# Autodesk Inventor assembly: assembled-feed
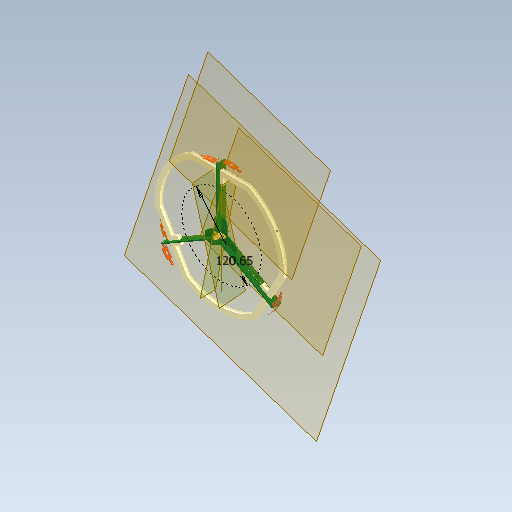
[picture p0: Inventor's stored thumbnail of the model, 512x512]
Saved by Autodesk Inventor 2021 (Build 250183000, 183)
## iProperties
Created: 2020-09-03
Part Number: assembled-feed
Document SubType Name: Assembly
Designer: dsouthall
Author: dsouthall
## Documents named in this file (4)
- C:\Users\dsouthall\OneDrive - The University of Chicago\Hpol\hpol-prototype\design\Model 8 in\assembled-feed.iam
- C:\Users\dsouthall\OneDrive - The University of Chicago\Hpol\hpol-prototype\design\Model 8 in\source\hub\tri-slot-hub.iam
- C:\Users\dsouthall\OneDrive - The University of Chicago\Hpol\hpol-prototype\design\Model 8 in\assembled-feed_feedline_8in.iam
- C:\Users\dsouthall\OneDrive - The University of Chicago\Hpol\hpol-prototype\design\Model 8 in\source\insert_8in.ipt
## Components (7 placed, 3 different names)
1. tri-slot-hub:1 [sub-assembly] — Mate:10, Angle:1, Mate:17, Mate:20, Mate:21, Mate:22, Mate:23, Mate:24, Mate:25, Mate:26, Mate:27, Mate:28, Mate:29, Mate:30
2. assembled-feed_feedline_8in:1 [sub-assembly] — Mate:21, Mate:22, Mate:23, Insert:4, Insert:6
3. assembled-feed_feedline_8in:2 [sub-assembly] — Mate:24, Mate:25, Mate:26, Insert:1, Insert:5
4. assembled-feed_feedline_8in:3 [sub-assembly] — Mate:27, Mate:28, Mate:29, Insert:2, Insert:3
5. insert_8in:1 — Insert:5, Insert:6
6. insert_8in:2 — Insert:1, Insert:2
7. insert_8in:3 — Insert:3, Insert:4
## Relationships (21: Mate 13, Insert 6, Angle 1, Flush 1)
- Mate:10: tri-slot-hub:1
- Angle:1 (0 deg): tri-slot-hub:1
- Mate:17: tri-slot-hub:1
- Mate:20: tri-slot-hub:1
- Flush:1 (-3.9973 mm)
- Mate:21: tri-slot-hub:1 ↔ assembled-feed_feedline_8in:1
- Mate:22: tri-slot-hub:1 ↔ assembled-feed_feedline_8in:1
- Mate:23: tri-slot-hub:1 ↔ assembled-feed_feedline_8in:1
- Mate:24: tri-slot-hub:1 ↔ assembled-feed_feedline_8in:2
- Mate:25: tri-slot-hub:1 ↔ assembled-feed_feedline_8in:2
- Mate:26: tri-slot-hub:1 ↔ assembled-feed_feedline_8in:2
- Mate:27: tri-slot-hub:1 ↔ assembled-feed_feedline_8in:3
- Mate:28: tri-slot-hub:1 ↔ assembled-feed_feedline_8in:3
- Mate:29: tri-slot-hub:1 ↔ assembled-feed_feedline_8in:3
- Mate:30 (-0.8 mm): tri-slot-hub:1
- Insert:1: assembled-feed_feedline_8in:2 ↔ insert_8in:2
- Insert:2: assembled-feed_feedline_8in:3 ↔ insert_8in:2
- Insert:3: assembled-feed_feedline_8in:3 ↔ insert_8in:3
- Insert:4: assembled-feed_feedline_8in:1 ↔ insert_8in:3
- Insert:5: assembled-feed_feedline_8in:2 ↔ insert_8in:1
- Insert:6: assembled-feed_feedline_8in:1 ↔ insert_8in:1
